# Autodesk Inventor assembly: DesignVer2(open)
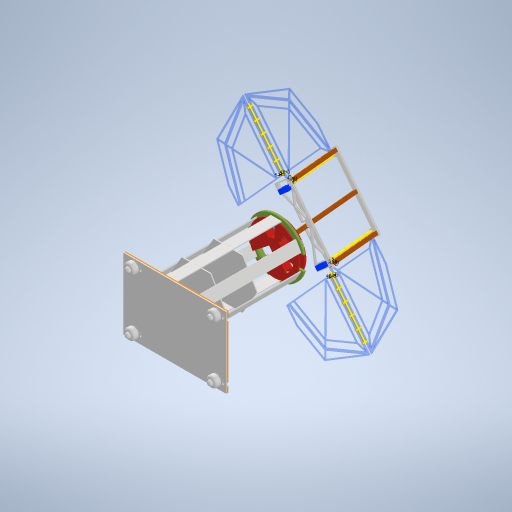
[picture p0: Inventor's stored thumbnail of the model, 512x512]
Saved by Autodesk Inventor 2024 (Build 280153000, 153)
## iProperties
Created: 2024-04-09
Part Number: DesignVer2(open)
Document SubType Name: Assembly
Designer: USER
Author: USER
## Documents named in this file (16)
- E:\university\大三\大三下\機工實務\圖檔\DesignVer2\DesignVer2(open).iam
- E:\university\大三\大三下\機工實務\圖檔\DesignVer2\base.ipt
- E:\university\大三\大三下\機工實務\圖檔\DesignVer2\cow_wheel.ipt
- E:\university\大三\大三下\機工實務\圖檔\DesignVer2\base_ver2.ipt
- E:\university\大三\大三下\機工實務\圖檔\DesignVer2\back_down_hold.ipt
- E:\university\大三\大三下\機工實務\圖檔\DesignVer2\back_cir_hold.ipt
- E:\university\大三\大三下\機工實務\圖檔\DesignVer2\middle_space.ipt
- E:\university\大三\大三下\機工實務\圖檔\DesignVer2\rolling_plate.ipt
- E:\university\大三\大三下\機工實務\圖檔\DesignVer2\rolling_plate_top.ipt
- E:\university\大三\大三下\機工實務\圖檔\DesignVer2\rolling_plate_small.ipt
- E:\university\大三\大三下\機工實務\圖檔\DesignVer2\左右.ipt
- E:\university\大三\大三下\機工實務\圖檔\DesignVer2\左右2.ipt
- E:\university\大三\大三下\機工實務\圖檔\DesignVer2\馬達.ipt
- E:\university\大三\大三下\機工實務\圖檔\DesignVer2\軸.ipt
- E:\university\大三\大三下\機工實務\圖檔\DesignVer2\螺絲.ipt
- E:\university\大三\大三下\機工實務\圖檔\DesignVer2\sail(open).iam
## Components (29 placed, 15 different names)
1. base:1 — 貼合:14, 齊平:3, 齊平:4, 貼合:15
2. cow_wheel:1
3. cow_wheel:2
4. cow_wheel:3
5. cow_wheel:4
6. base_ver2:1 — 貼合:16, 貼合:17, 貼合:18, 貼合:19, 貼合:24, 貼合:25, 貼合:26, 貼合:27, 貼合:37, 貼合:38, 貼合:39, 貼合:40, 貼合:72
7. back_down_hold:1 — 齊平:7, 齊平:8, 齊平:9, 貼合:39, 貼合:40, 相切:2
8. back_down_hold:2 — 貼合:18, 貼合:19, 貼合:34, 齊平:14, 相切:1, 貼合:72, 齊平:28
9. back_down_hold:3 — 齊平:5, 貼合:26, 貼合:27, 貼合:47, 齊平:13
10. back_down_hold:4 — 齊平:8, 齊平:9, 貼合:37, 貼合:38
11. back_down_hold:5 — 齊平:6, 齊平:7, 貼合:24, 貼合:25, 貼合:46, 齊平:12, 貼合:48
12. back_down_hold:6 — 齊平:5, 齊平:6, 貼合:15, 貼合:16, 貼合:17, 貼合:32, 貼合:33
13. back_cir_hold:1 — 貼合:32, 貼合:33, 貼合:34, 貼合:51
14. middle_space:1 — 齊平:13, 貼合:48, 齊平:14, 齊平:28
15. middle_space:2 — 貼合:46, 齊平:12, 貼合:47
16. rolling_plate:1 — 貼合:49, 貼合:50, 齊平:15, 貼合:51, 貼合:55, 齊平:22, 齊平:23
17. rolling_plate:2 — 貼合:56, 貼合:57, 齊平:24
18. rolling_plate_top:1 — 貼合:49, 貼合:50, 齊平:15, 相切:1, 相切:2, 貼合:58, 貼合:59, 貼合:60, 貼合:61, 貼合:62, 貼合:63
19. rolling_plate_small:1 — 貼合:52, 齊平:16, 齊平:19, 貼合:56, 齊平:24
20. rolling_plate_small:2 — 貼合:52, 貼合:53, 齊平:16, 齊平:17, 齊平:19, 齊平:20, 貼合:57
21. rolling_plate_small:3 — 貼合:53, 貼合:54, 齊平:17, 齊平:18, 齊平:20, 齊平:21
22. rolling_plate_small:4 — 貼合:54, 齊平:18, 齊平:21, 貼合:55, 齊平:22, 齊平:23
23. 左右:1 — 貼合:58, 貼合:59, 貼合:60, 貼合:66, 貼合:67, 齊平:26, 貼合:68, 齊平:27
24. 左右2:1 — 貼合:61, 貼合:62, 貼合:63
25. 馬達:1 — 貼合:64, 貼合:65, 貼合:69, 貼合:70, 貼合:71
26. 軸:1 — 貼合:64, 貼合:65, 貼合:73, 貼合:74, 貼合:75
27. 螺絲:1 — 齊平:25, 貼合:66, 貼合:67, 齊平:26, 貼合:69, 貼合:70
28. 螺絲:2 — 齊平:25, 貼合:68, 齊平:27, 貼合:71
29. sail(open):1 [sub-assembly] — 貼合:73, 貼合:74, 貼合:75
## Relationships (88: Mate 60, Flush 26, Tangent 2)
- [Mate]: base:1 ↔ cow_wheel:4
- [Mate]: base:1 ↔ cow_wheel:4
- [Mate]: base:1 ↔ cow_wheel:4
- [Mate]: base:1 ↔ cow_wheel:3
- [Mate]: base:1 ↔ cow_wheel:3
- [Mate]: base:1 ↔ cow_wheel:3
- [Mate]: base:1 ↔ cow_wheel:2
- [Mate]: base:1 ↔ cow_wheel:2
- [Mate]: base:1 ↔ cow_wheel:1
- [Mate]: base:1 ↔ cow_wheel:1
- [Mate]: base:1 ↔ cow_wheel:2
- [Mate]: base:1 ↔ cow_wheel:1
- [Mate]: base:1 ↔ base_ver2:1
- [Flush]: base:1 ↔ base_ver2:1
- [Flush]: base:1 ↔ base_ver2:1
- 貼合:14 [Mate]: base:1
- 齊平:3 [Flush]: base:1
- 齊平:4 [Flush]: base:1
- 齊平:5 [Flush]: back_down_hold:3 ↔ back_down_hold:6
- 齊平:6 [Flush]: back_down_hold:5 ↔ back_down_hold:6
- 齊平:7 [Flush]: back_down_hold:1 ↔ back_down_hold:5
- 齊平:8 [Flush]: back_down_hold:1 ↔ back_down_hold:4
- 貼合:15 [Mate]: base:1 ↔ back_down_hold:6
- 貼合:16 [Mate]: base_ver2:1 ↔ back_down_hold:6
- 貼合:17 [Mate]: base_ver2:1 ↔ back_down_hold:6
- 貼合:18 [Mate]: base_ver2:1 ↔ back_down_hold:2
- 貼合:19 [Mate]: base_ver2:1 ↔ back_down_hold:2
- 貼合:24 [Mate]: base_ver2:1 ↔ back_down_hold:5
- 貼合:25 [Mate]: base_ver2:1 ↔ back_down_hold:5
- 貼合:26 [Mate]: base_ver2:1 ↔ back_down_hold:3
- 貼合:27 [Mate]: base_ver2:1 ↔ back_down_hold:3
- 齊平:9 [Flush]: back_down_hold:1 ↔ back_down_hold:4
- 貼合:32 [Mate]: back_down_hold:6 ↔ back_cir_hold:1
- 貼合:33 [Mate]: back_down_hold:6 ↔ back_cir_hold:1
- 貼合:34 [Mate]: back_down_hold:2 ↔ back_cir_hold:1
- 貼合:37 [Mate]: base_ver2:1 ↔ back_down_hold:4
- 貼合:38 [Mate]: base_ver2:1 ↔ back_down_hold:4
- 貼合:39 [Mate]: base_ver2:1 ↔ back_down_hold:1
- 貼合:40 [Mate]: base_ver2:1 ↔ back_down_hold:1
- 貼合:46 [Mate]: back_down_hold:5 ↔ middle_space:2
- 齊平:12 [Flush]: back_down_hold:5 ↔ middle_space:2
- 貼合:47 [Mate]: back_down_hold:3 ↔ middle_space:2
- 齊平:13 [Flush]: back_down_hold:3 ↔ middle_space:1
- 貼合:48 [Mate]: back_down_hold:5 ↔ middle_space:1
- 齊平:14 [Flush]: back_down_hold:2 ↔ middle_space:1
- 貼合:49 [Mate]: rolling_plate:1 ↔ rolling_plate_top:1
- 貼合:50 [Mate]: rolling_plate:1 ↔ rolling_plate_top:1
- 齊平:15 [Flush]: rolling_plate:1 ↔ rolling_plate_top:1
- 貼合:51 [Mate] (0.5 mm): back_cir_hold:1 ↔ rolling_plate:1
- 相切:1 [Tangent]: back_down_hold:2 ↔ rolling_plate_top:1
- 相切:2 [Tangent]: back_down_hold:1 ↔ rolling_plate_top:1
- 貼合:52 [Mate]: rolling_plate_small:1 ↔ rolling_plate_small:2
- 貼合:53 [Mate]: rolling_plate_small:2 ↔ rolling_plate_small:3
- 貼合:54 [Mate]: rolling_plate_small:3 ↔ rolling_plate_small:4
- 齊平:16 [Flush]: rolling_plate_small:1 ↔ rolling_plate_small:2
- 齊平:17 [Flush]: rolling_plate_small:2 ↔ rolling_plate_small:3
- 齊平:18 [Flush]: rolling_plate_small:3 ↔ rolling_plate_small:4
- 齊平:19 [Flush]: rolling_plate_small:1 ↔ rolling_plate_small:2
- 齊平:20 [Flush]: rolling_plate_small:2 ↔ rolling_plate_small:3
- 齊平:21 [Flush]: rolling_plate_small:3 ↔ rolling_plate_small:4
- 貼合:55 [Mate]: rolling_plate:1 ↔ rolling_plate_small:4
- 齊平:22 [Flush]: rolling_plate:1 ↔ rolling_plate_small:4
- 齊平:23 [Flush]: rolling_plate:1 ↔ rolling_plate_small:4
- 貼合:56 [Mate]: rolling_plate:2 ↔ rolling_plate_small:1
- 貼合:57 [Mate]: rolling_plate:2 ↔ rolling_plate_small:2
- 齊平:24 [Flush]: rolling_plate:2 ↔ rolling_plate_small:1
- 貼合:58 [Mate]: rolling_plate_top:1 ↔ 左右:1
- 貼合:59 [Mate]: rolling_plate_top:1 ↔ 左右:1
- 貼合:60 [Mate]: rolling_plate_top:1 ↔ 左右:1
- 貼合:61 [Mate]: rolling_plate_top:1 ↔ 左右2:1
- 貼合:62 [Mate]: rolling_plate_top:1 ↔ 左右2:1
- 貼合:63 [Mate]: rolling_plate_top:1 ↔ 左右2:1
- 貼合:64 [Mate]: 馬達:1 ↔ 軸:1
- 貼合:65 [Mate]: 馬達:1 ↔ 軸:1
- 齊平:25 [Flush]: 螺絲:1 ↔ 螺絲:2
- 貼合:66 [Mate]: 左右:1 ↔ 螺絲:1
- 貼合:67 [Mate]: 左右:1 ↔ 螺絲:1
- 齊平:26 [Flush]: 左右:1 ↔ 螺絲:1
- 貼合:68 [Mate]: 左右:1 ↔ 螺絲:2
- 齊平:27 [Flush]: 左右:1 ↔ 螺絲:2
- 貼合:69 [Mate]: 馬達:1 ↔ 螺絲:1
- 貼合:70 [Mate]: 馬達:1 ↔ 螺絲:1
- 貼合:71 [Mate]: 馬達:1 ↔ 螺絲:2
- 貼合:72 [Mate]: base_ver2:1 ↔ back_down_hold:2
- 齊平:28 [Flush]: back_down_hold:2 ↔ middle_space:1
- 貼合:73 [Mate]: 軸:1 ↔ sail(open):1
- 貼合:74 [Mate]: 軸:1 ↔ sail(open):1
- 貼合:75 [Mate]: 軸:1 ↔ sail(open):1
